# Autodesk Inventor assembly: TEAM 6 UPDATED ASSEMBLY
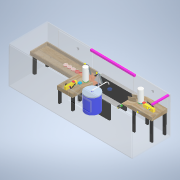
[picture p0: Inventor's stored thumbnail of the model, 180x180]
Saved by Autodesk Inventor 2021 (Build 250183000, 183)
## iProperties
Created: 2021-07-09
Part Number: TEAM 6 UPDATED ASSEMBLY
Document SubType Name: Assembly
Designer: HP
Author: HP
## Documents named in this file (45)
- C:\Users\HP\Documents\TEAM 6 UPDATED ASSEMBLY.iam
- C:\Users\HP\Documents\CONTAINER NEW.ipt
- C:\Users\HP\Downloads\pole.ipt
- C:\Users\HP\Documents\CONTAINER PIPE.ipt
- C:\Users\HP\Documents\SENSOR.ipt
- C:\Users\HP\Documents\TABLE NEW.ipt
- C:\Users\HP\Documents\DC SUBMERSIBLE PUMP.ipt
- C:\Users\HP\Documents\PETRI DISH.ipt
- C:\Users\HP\Downloads\pouring part 123.ipt
- C:\Users\HP\Documents\LID NEW UPDATED.ipt
- C:\Users\HP\Documents\STACK NEW..ipt
- C:\Users\HP\Documents\CAP.ipt
- C:\Users\HP\Documents\CAP PROCESS SKETCH.ipt
- C:\Users\HP\Documents\WOODEN CORRECT SLIDER.ipt
- C:\Users\HP\Documents\TABLE FOR VERTI.ipt
- C:\Users\HP\Documents\SLIDERCRANK-BASE CUBOID.ipt
- C:\Users\HP\Documents\SLIDER CRANK-ROLL.ipt
- C:\Users\HP\Documents\SLIDER CRANK-FIRST REVOLUTER.ipt
- C:\Users\HP\Documents\SLIDER CRANK LONG BAR.ipt
- C:\Users\HP\Documents\SLIDER CRANK PUSHER.ipt
- C:\Users\HP\Documents\ASSEMBLED BOX EXTRUDE1.ipt
- C:\Users\HP\Documents\SC BOLT.ipt
- C:\Users\HP\Documents\SC DC MOTOR.ipt
- C:\Users\HP\Documents\BELT.ipt
- C:\Users\HP\Documents\BOLT 3.ipt
- C:\Users\HP\Documents\BOLT4.ipt
- C:\Users\HP\Documents\push for plate.ipt
- C:\Users\HP\Documents\Part9.ipt
- C:\Users\HP\Documents\Part10.ipt
- C:\Users\HP\Documents\uv environment.ipt
- C:\Users\HP\Documents\UV.ipt
- C:\Users\HP\Documents\uv2.ipt
- C:\Users\HP\Documents\Part5.ipt
- C:\Users\HP\Documents\BELT WOOD SUPPORT.ipt
- C:\Users\HP\Documents\conveyor stand.ipt
- C:\Users\HP\Documents\conveyor roller.ipt
- C:\Users\HP\Documents\Part8.ipt
- C:\Users\HP\Documents\bolt6.ipt
- C:\Users\HP\Documents\stand1.ipt
- C:\Users\HP\Documents\another closed side.ipt
- C:\Users\HP\Documents\closed side3.ipt
- C:\Users\HP\Documents\Part3.ipt
- C:\Users\HP\Documents\lid1.ipt
- C:\Users\HP\Documents\lid2.ipt
- C:\Users\HP\Documents\lid3.ipt
## Components (81 placed, 44 different names)
1. CONTAINER NEW:1
2. pole:1
3. CONTAINER PIPE:1
4. SENSOR:3
5. TABLE NEW:1 — Flush:13
6. DC SUBMERSIBLE PUMP:1
7. PETRI DISH:3
8. PETRI DISH:6
9. PETRI DISH:7
10. PETRI DISH:9
11. PETRI DISH:10
12. PETRI DISH:11
13. PETRI DISH:12
14. PETRI DISH:13
15. PETRI DISH:14
16. PETRI DISH:15
17. PETRI DISH:16 — Cylindrical:1, Slider:3, Angle:3
18. pouring part 123:1
19. LID NEW UPDATED:1
20. STACK NEW.:1
21. SENSOR:4
22. CAP PROCESS SKETCH:1
23. TABLE NEW:2
24. WOODEN CORRECT SLIDER:1
25. STACK NEW.:3 — Flush:5
26. CAP:2
27. pole:2
28. SENSOR:5
29. TABLE FOR VERTI:1 — Flush:9
30. PETRI DISH:20
31. CAP:5
32. pouring part 123:2
33. PETRI DISH:21
34. PETRI DISH:22
35. PETRI DISH:23
36. PETRI DISH:24
37. CAP:7
38. CAP:8
39. CAP:9
40. SLIDERCRANK-BASE CUBOID:1 — Mate:1, Slider:1, Flush:1, Angle:1, Flush:7, Flush:8
41. SLIDER CRANK-ROLL:1 — Mate:1, Mate:2
42. SLIDER CRANK-FIRST REVOLUTER:1 — Mate:2, Mate:3, Mate:5, Angle:1
43. SLIDER CRANK LONG BAR:1 — Mate:3, Mate:4, Mate:5, Mate:6
44. SLIDER CRANK PUSHER:1 — Slider:1, Mate:4, Mate:7
45. ASSEMBLED BOX EXTRUDE1:1 — Flush:1
46. SC BOLT:1 — Mate:6
47. SC BOLT:2 — Mate:7
48. SC DC MOTOR:1 — Flush:19
49. BELT:1 — Mate:16, Mate:17
50. SLIDERCRANK-BASE CUBOID:2 — Mate:8, Slider:2, Angle:2, Flush:6, Mate:18
51. SLIDER CRANK-FIRST REVOLUTER:2 — Mate:9, Flush:2, Mate:10, Mate:11, Angle:2
52. SLIDER CRANK-ROLL:2 — Mate:8, Mate:9, Flush:2
53. SLIDER CRANK LONG BAR:2 — Mate:10, Mate:11, Mate:12, Mate:13, Flush:4, Mate:15
54. SLIDER CRANK PUSHER:2 — Slider:2, Mate:12, Mate:13, Flush:3, Mate:14
55. BOLT 3:1 — Flush:3, Mate:14
56. BOLT4:1 — Flush:4, Mate:15
57. push for plate:1 — Flush:5
58. Part9:1 — Flush:6
59. Part10:1 — Flush:7, Flush:8
60. uv environment:1 — Flush:9, Flush:10, Flush:11, Flush:12, Flush:20, Flush:21, Flush:22, Flush:23, Flush:24
61. UV:1 — Flush:10
62. uv2:1 — Flush:11, Flush:12
63. CAP:10 — Cylindrical:1, Slider:3, Angle:3
64. Part5:1 — Flush:13
65. BELT WOOD SUPPORT:1 — Flush:14, Flush:15
66. conveyor stand:1 — Flush:14, Flush:15
67. conveyor roller:1 — Mate:16, Flush:16, Flush:17
68. conveyor roller:2 — Mate:17
69. Part8:1 — Flush:16, Flush:17, Flush:18
70. bolt6:1 — Flush:18
71. SC DC MOTOR:2
72. stand1:1 — Flush:19
73. SC DC MOTOR:3 — Mate:18
74. Part8:2
75. bolt6:2
76. another closed side:1 — Flush:20, Flush:21, Flush:22, Flush:25, Flush:26
77. closed side3:1 — Flush:23, Flush:24
78. Part3:1 — Flush:25, Flush:26
79. lid1:1
80. lid2:1
81. lid3:1
## Relationships (51: Flush 26, Mate 18, TranslationJoint 3, Angle 3, CylindricalJoint 1)
- Mate:1: SLIDERCRANK-BASE CUBOID:1 ↔ SLIDER CRANK-ROLL:1
- Mate:2: SLIDER CRANK-ROLL:1 ↔ SLIDER CRANK-FIRST REVOLUTER:1
- Mate:3: SLIDER CRANK-FIRST REVOLUTER:1 ↔ SLIDER CRANK LONG BAR:1
- Slider:1 [TranslationJoint]: SLIDERCRANK-BASE CUBOID:1 ↔ SLIDER CRANK PUSHER:1
- Mate:4: SLIDER CRANK LONG BAR:1 ↔ SLIDER CRANK PUSHER:1
- Flush:1: SLIDERCRANK-BASE CUBOID:1 ↔ ASSEMBLED BOX EXTRUDE1:1
- Mate:5: SLIDER CRANK-FIRST REVOLUTER:1 ↔ SLIDER CRANK LONG BAR:1
- Mate:6: SLIDER CRANK LONG BAR:1 ↔ SC BOLT:1
- Mate:7: SLIDER CRANK PUSHER:1 ↔ SC BOLT:2
- Angle:1 (1248 deg): SLIDERCRANK-BASE CUBOID:1 ↔ SLIDER CRANK-FIRST REVOLUTER:1
- Mate:8: SLIDERCRANK-BASE CUBOID:2 ↔ SLIDER CRANK-ROLL:2
- Mate:9: SLIDER CRANK-FIRST REVOLUTER:2 ↔ SLIDER CRANK-ROLL:2
- Flush:2: SLIDER CRANK-FIRST REVOLUTER:2 ↔ SLIDER CRANK-ROLL:2
- Mate:10: SLIDER CRANK-FIRST REVOLUTER:2 ↔ SLIDER CRANK LONG BAR:2
- Mate:11: SLIDER CRANK-FIRST REVOLUTER:2 ↔ SLIDER CRANK LONG BAR:2
- Slider:2 [TranslationJoint]: SLIDERCRANK-BASE CUBOID:2 ↔ SLIDER CRANK PUSHER:2
- Mate:12: SLIDER CRANK LONG BAR:2 ↔ SLIDER CRANK PUSHER:2
- Mate:13: SLIDER CRANK LONG BAR:2 ↔ SLIDER CRANK PUSHER:2
- Angle:2 (1627 deg): SLIDERCRANK-BASE CUBOID:2 ↔ SLIDER CRANK-FIRST REVOLUTER:2
- Flush:3: SLIDER CRANK PUSHER:2 ↔ BOLT 3:1
- Mate:14: SLIDER CRANK PUSHER:2 ↔ BOLT 3:1
- Flush:4: SLIDER CRANK LONG BAR:2 ↔ BOLT4:1
- Mate:15: SLIDER CRANK LONG BAR:2 ↔ BOLT4:1
- Flush:5: STACK NEW.:3 ↔ push for plate:1
- Flush:6: SLIDERCRANK-BASE CUBOID:2 ↔ Part9:1
- Flush:7: SLIDERCRANK-BASE CUBOID:1 ↔ Part10:1
- Flush:8: SLIDERCRANK-BASE CUBOID:1 ↔ Part10:1
- Flush:9: TABLE FOR VERTI:1 ↔ uv environment:1
- Flush:10: uv environment:1 ↔ UV:1
- Flush:11: uv environment:1 ↔ uv2:1
- Flush:12: uv environment:1 ↔ uv2:1
- Cylindrical:1: PETRI DISH:16 ↔ CAP:10
- Slider:3 [TranslationJoint]: PETRI DISH:16 ↔ CAP:10
- Angle:3 (0 deg): PETRI DISH:16 ↔ CAP:10
- Flush:13: TABLE NEW:1 ↔ Part5:1
- Flush:14: BELT WOOD SUPPORT:1 ↔ conveyor stand:1
- Flush:15: BELT WOOD SUPPORT:1 ↔ conveyor stand:1
- Mate:16: BELT:1 ↔ conveyor roller:1
- Mate:17: BELT:1 ↔ conveyor roller:2
- Flush:16: conveyor roller:1 ↔ Part8:1
- Flush:17: conveyor roller:1 ↔ Part8:1
- Flush:18: Part8:1 ↔ bolt6:1
- Flush:19: SC DC MOTOR:1 ↔ stand1:1
- Mate:18: SLIDERCRANK-BASE CUBOID:2 ↔ SC DC MOTOR:3
- Flush:20: uv environment:1 ↔ another closed side:1
- Flush:21: uv environment:1 ↔ another closed side:1
- Flush:22: uv environment:1 ↔ another closed side:1
- Flush:23: uv environment:1 ↔ closed side3:1
- Flush:24: uv environment:1 ↔ closed side3:1
- Flush:25: another closed side:1 ↔ Part3:1
- Flush:26: another closed side:1 ↔ Part3:1
